# Autodesk Inventor assembly: Wing Left
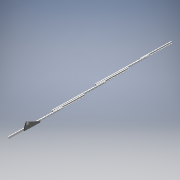
[picture p0: Inventor's stored thumbnail of the model, 180x180]
Saved by Autodesk Inventor 2019 (Build 230136000, 136)
## iProperties
Part Number: Wing Left
Document SubType Name: Assembly
Designer: Delta
Author: Delta
## Documents named in this file (5)
- C:\Robotics\CAD\2019-20_CAD\Collection\Wing Left.iam
- C:\Robotics\CAD\2019-20_CAD\Collection\Triangle axle slide connector.ipt
- C:\Robotics\CAD\COTSParts\Rev\REV-41-1683 Bear Blocks.ipt
- C:\Robotics\CAD\COTSParts\Misumi_Slides\AIS2018\SAR330.iam
- C:\Robotics\CAD\2018-19_CAD\2019-20_CAD\offseason\slide conector.ipt
## Components (7 placed, 4 different names)
1. Triangle axle slide connector:1 — Mate:3, Angle:1, Mate:4, Mate:5, Mate:6
2. REV-41-1683 Bear Blocks:1 — Mate:3, Angle:1
3. slide conector:1 — Mate:7, Mate:8, Mate:9, Mate:10, Mate:11, Mate:12
4. slide conector:2 — Mate:13, Mate:14, Mate:15, Mate:16, Mate:17, Mate:18
5. SAR330:1 [sub-assembly] — Mate:16, Mate:17, Mate:18
6. SAR330:2 [sub-assembly] — Mate:10, Mate:11, Mate:12, Mate:13, Mate:14, Mate:15
7. SAR330:3 [sub-assembly] — Mate:4, Mate:5, Mate:6, Mate:7, Mate:8, Mate:9
## Relationships (17: Mate 16, Angle 1)
- Mate:3: Triangle axle slide connector:1 ↔ REV-41-1683 Bear Blocks:1
- Angle:1 (0 deg): Triangle axle slide connector:1 ↔ REV-41-1683 Bear Blocks:1
- Mate:4: Triangle axle slide connector:1 ↔ SAR330:3
- Mate:5: Triangle axle slide connector:1 ↔ SAR330:3
- Mate:6: Triangle axle slide connector:1 ↔ SAR330:3
- Mate:7: slide conector:1 ↔ SAR330:3
- Mate:8: slide conector:1 ↔ SAR330:3
- Mate:9: slide conector:1 ↔ SAR330:3
- Mate:10: slide conector:1 ↔ SAR330:2
- Mate:11: slide conector:1 ↔ SAR330:2
- Mate:12: slide conector:1 ↔ SAR330:2
- Mate:13: slide conector:2 ↔ SAR330:2
- Mate:14: slide conector:2 ↔ SAR330:2
- Mate:15: slide conector:2 ↔ SAR330:2
- Mate:16: slide conector:2 ↔ SAR330:1
- Mate:17: slide conector:2 ↔ SAR330:1
- Mate:18: slide conector:2 ↔ SAR330:1
